# Autodesk Inventor assembly: AssemblyUpdated
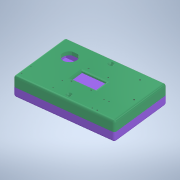
[picture p0: Inventor's stored thumbnail of the model, 180x180]
Saved by Autodesk Inventor 2022.3 (Build 263350000, 350)
## iProperties
Created: 2023-06-27
Part Number: AssemblyUpdated
Document SubType Name: Assembly
Designer: natalie.jimenez
Author: natalie.jimenez
## Documents named in this file (4)
- C:\Users\natalie.jimenez\Desktop\AssemblyUpdated.iam
- C:\Users\natalie.jimenez\Desktop\Prototype.ipt
- C:\Users\natalie.jimenez\Desktop\PrototypeBack.ipt
- C:\Users\natalie.jimenez\Desktop\Strap_RS485.ipt
## Components (3 placed, 3 different names)
1. Prototype:1 — Mate:1, Mate:2, Mate:3, Mate:4, Mate:5
2. PrototypeBack:1 — Mate:1, Mate:4, Mate:5
3. Strap_RS485:1 — Mate:2, Mate:3
## Relationships (5: Mate 5)
- Mate:1: Prototype:1 ↔ PrototypeBack:1
- Mate:2: Prototype:1 ↔ Strap_RS485:1
- Mate:3: Prototype:1 ↔ Strap_RS485:1
- Mate:4: Prototype:1 ↔ PrototypeBack:1
- Mate:5: Prototype:1 ↔ PrototypeBack:1
